# Autodesk Inventor assembly: Vehicle Registration Plate
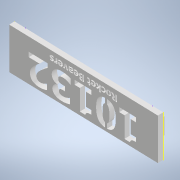
[picture p0: Inventor's stored thumbnail of the model, 180x180]
Saved by Autodesk Inventor 2020 (Build 240168000, 168)
## iProperties
Created: 2020-01-17
Part Number: Vehicle Registration Plate
Document SubType Name: Assembly
Designer: maple
Author: maple
## Documents named in this file (3)
- C:\Users\maple\Documents\GitHub\3D-Models\Robotics\Vehicle Registration Plate.iam
- C:\Users\maple\Documents\GitHub\3D-Models\Robotics\Vehicle Registration Plate.ipt
- C:\Users\maple\Documents\GitHub\3D-Models\Robotics\Mount Male.ipt
## Components (3 placed, 2 different names)
1. Vehicle Registration Plate:1 — Rigid:1, Rigid:2
2. Mount Male:1 — Rigid:2
3. Mount Male:2 — Rigid:1
## Relationships (2: WeldJoint 2)
- Rigid:1 [WeldJoint]: Vehicle Registration Plate:1 ↔ Mount Male:2
- Rigid:2 [WeldJoint]: Vehicle Registration Plate:1 ↔ Mount Male:1
